# Autodesk Inventor assembly: Assembly_Cube_CircularAperture_v3
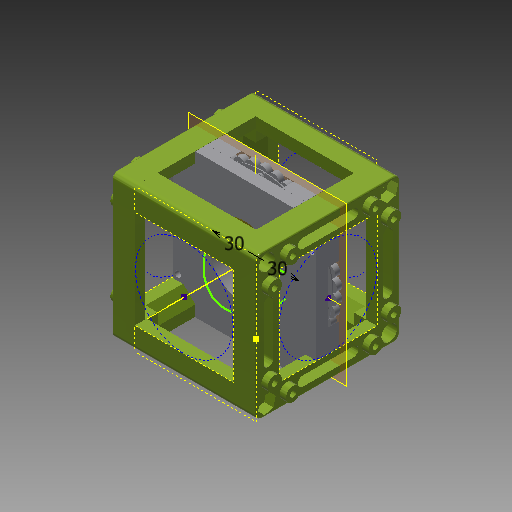
[picture p0: Inventor's stored thumbnail of the model, 512x512]
Saved by Autodesk Inventor 2019 (Build 230136000, 136)
## iProperties
Created: 2019-10-23
Part Number: Assembly_Cube_CircularAperture_v3
Document SubType Name: Assembly
Designer: marsikovabarbora
Author: marsikovabarbora
## Documents named in this file (6)
- C:\Users\marsikovabarbora\Dropbox\UC2\02_CAD\INVENTOR\uc2_v3\Assembly_Cube_CircularAperture_v3.iam
- C:\Users\marsikovabarbora\Dropbox\UC2\02_CAD\INVENTOR\uc2_v3\20_Cube_Insert_CirAp_Lid_v3.ipt
- C:\Users\marsikovabarbora\Dropbox\UC2\02_CAD\INVENTOR\uc2_v3\20_Cube_Insert_CirAp_Wheel.ipt
- C:\Users\marsikovabarbora\Dropbox\UC2\02_CAD\INVENTOR\uc2_v3\20_Cube_Insert_CirAp_Leaf.ipt
- C:\Users\marsikovabarbora\Dropbox\UC2\02_CAD\INVENTOR\uc2_v3\20_Cube_Insert_CirAp_Guide_v3.ipt
- C:\Users\marsikovabarbora\Dropbox\UC2\02_CAD\INVENTOR\uc2_v3\Assembly_Cube_empty_IM_v3.iam
## Components (11 placed, 5 different names)
1. 20_Cube_Insert_CirAp_Lid_v3:1 — Flush:2, Mate:6, Angle:2
2. 20_Cube_Insert_CirAp_Wheel:1 — Flush:2, Flush:3, Flush:4, Mate:5
3. 20_Cube_Insert_CirAp_Guide_v3:1 — Mate:6, Angle:2, Passend:7, Winkel:3, Passend:8
4. Assembly_Cube_empty_IM_v3:1 [sub-assembly] — Passend:7, Winkel:3, Passend:8
5. 20_Cube_Insert_CirAp_Leaf:1 — Flush:3, Flush:4, Mate:5
6. 20_Cube_Insert_CirAp_Leaf:2
7. 20_Cube_Insert_CirAp_Leaf:3
8. 20_Cube_Insert_CirAp_Leaf:4
9. 20_Cube_Insert_CirAp_Leaf:5
10. 20_Cube_Insert_CirAp_Leaf:6
11. 20_Cube_Insert_CirAp_Leaf:7
## Component patterns: (7 elements, first: 20_Cube_Insert_CirAp_Leaf:1)
## Relationships (9: Mate 4, Flush 3, Angle 2)
- Flush:2: 20_Cube_Insert_CirAp_Lid_v3:1 ↔ 20_Cube_Insert_CirAp_Wheel:1
- Flush:3: 20_Cube_Insert_CirAp_Wheel:1 ↔ 20_Cube_Insert_CirAp_Leaf:1
- Flush:4: 20_Cube_Insert_CirAp_Wheel:1 ↔ 20_Cube_Insert_CirAp_Leaf:1
- Mate:5: 20_Cube_Insert_CirAp_Wheel:1 ↔ 20_Cube_Insert_CirAp_Leaf:1
- Mate:6: 20_Cube_Insert_CirAp_Lid_v3:1 ↔ 20_Cube_Insert_CirAp_Guide_v3:1
- Angle:2 (0 deg): 20_Cube_Insert_CirAp_Lid_v3:1 ↔ 20_Cube_Insert_CirAp_Guide_v3:1
- Passend:7 [Mate]: 20_Cube_Insert_CirAp_Guide_v3:1 ↔ Assembly_Cube_empty_IM_v3:1
- Winkel:3 [Angle] (0 deg): 20_Cube_Insert_CirAp_Guide_v3:1 ↔ Assembly_Cube_empty_IM_v3:1
- Passend:8 [Mate]: 20_Cube_Insert_CirAp_Guide_v3:1 ↔ Assembly_Cube_empty_IM_v3:1
